# Autodesk Inventor assembly: ASY ANP 1490 FDS one way
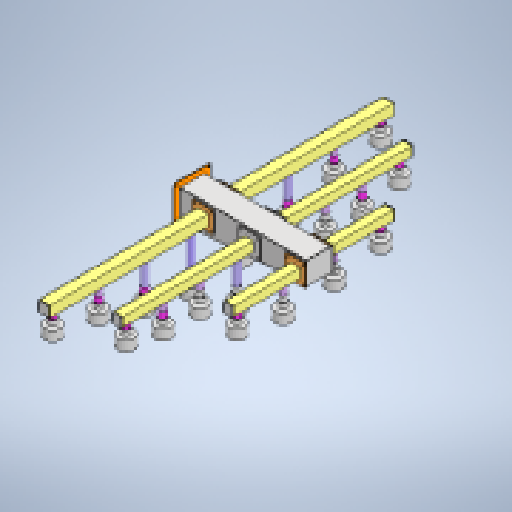
[picture p0: Inventor's stored thumbnail of the model, 512x512]
Saved by Autodesk Inventor 2025.3 (Build 293356030, 356C)
## iProperties
Created: 2025-07-22
Part Number: ASY ANP 1490 FDS one way
Document SubType Name: Assembly
Designer: admin
Stock Number: 20x40
Author: admin
## Documents named in this file (8)
- C:\Users\admin\Yandex.Disk\home pc\Inventor\ANP--Antipayuta\FDS 1400\ASY ANP 1490 FDS one way.iam
- C:\Users\admin\Yandex.Disk\home pc\Inventor\ANP--Antipayuta\FDS 1400\ANP 1422 BOTTOM FDS diameter way up.ipt
- C:\Users\admin\Yandex.Disk\home pc\Inventor\ANP--Antipayuta\FDS 1400\ANP 1421 FDS Diam way flange 1.ipt
- C:\Users\admin\Yandex.Disk\home pc\Inventor\ANP--Antipayuta\FDS 1400\ANP 1423 BOTTOM FDS diameter way down.ipt
- C:\Users\admin\Yandex.Disk\home pc\Inventor\ANP--Antipayuta\FDS 1400\ASY ANP 1425 FDS way 5.iam
- C:\Users\admin\Yandex.Disk\home pc\Inventor\ANP--Antipayuta\FDS 1400\ASY ANP 1426 FDS way 6.iam
- C:\Users\admin\Yandex.Disk\home pc\Inventor\ANP--Antipayuta\FDS 1400\ASY ANP 1427 FDS way 7.iam
- C:\Users\admin\Yandex.Disk\home pc\Inventor\ANP--Antipayuta\FDS 1400\ANP 1424 FDS diam way cup.ipt
## Components (10 placed, 10 different names)
1. ANP 1422 BOTTOM FDS diameter way up.ipt:1 — Rigid:21, Rigid:25, Rigid:26
2. ANP 1421 FDS Diam way flange 1.ipt:1
3. ANP 1423 BOTTOM FDS diameter way down.ipt:1 — Rigid:18, Rigid:22, Rigid:27, Rotational:1
4. ASY ANP 1425 FDS way 5.iam:1 [sub-assembly] — Rigid:21
5. ASY ANP 1426 FDS way 6.iam:1 [sub-assembly] — Rigid:25
6. ASY ANP 1427 FDS way 7.iam:1 [sub-assembly] — Rigid:26
7. ANP 1424 FDS diam way cup.ipt:1 — Rigid:18
8. ASY ANP 1425 FDS way 5:2 [sub-assembly] — Rigid:22
9. ASY ANP 1426 FDS way 6:2 [sub-assembly] — Rigid:27
10. ASY ANP 1427 FDS way 7:2 [sub-assembly] — Rotational:1
## Relationships (13: WeldJoint 6, Mate 3, Flush 3, RevoluteJoint 1)
- [Mate]: ANP 1422 BOTTOM FDS diameter way up.ipt:1 ↔ ANP 1421 FDS Diam way flange 1.ipt:1
- [Flush]: ANP 1422 BOTTOM FDS diameter way up.ipt:1 ↔ ANP 1421 FDS Diam way flange 1.ipt:1
- [Flush]: ANP 1422 BOTTOM FDS diameter way up.ipt:1 ↔ ANP 1421 FDS Diam way flange 1.ipt:1
- [Mate]: ANP 1421 FDS Diam way flange 1.ipt:1 ↔ ANP 1423 BOTTOM FDS diameter way down.ipt:1
- [Flush]: ANP 1421 FDS Diam way flange 1.ipt:1 ↔ ANP 1423 BOTTOM FDS diameter way down.ipt:1
- [Mate]: ANP 1422 BOTTOM FDS diameter way up.ipt:1 ↔ ANP 1423 BOTTOM FDS diameter way down.ipt:1
- Rigid:18 [WeldJoint]: ANP 1423 BOTTOM FDS diameter way down.ipt:1 ↔ ANP 1424 FDS diam way cup.ipt:1
- Rigid:21 [WeldJoint]: ANP 1422 BOTTOM FDS diameter way up.ipt:1 ↔ ASY ANP 1425 FDS way 5.iam:1
- Rigid:22 [WeldJoint]: ANP 1423 BOTTOM FDS diameter way down.ipt:1 ↔ ASY ANP 1425 FDS way 5:2
- Rigid:25 [WeldJoint]: ANP 1422 BOTTOM FDS diameter way up.ipt:1 ↔ ASY ANP 1426 FDS way 6.iam:1
- Rigid:26 [WeldJoint]: ANP 1422 BOTTOM FDS diameter way up.ipt:1 ↔ ASY ANP 1427 FDS way 7.iam:1
- Rigid:27 [WeldJoint]: ANP 1423 BOTTOM FDS diameter way down.ipt:1 ↔ ASY ANP 1426 FDS way 6:2
- Rotational:1 [RevoluteJoint]: ANP 1423 BOTTOM FDS diameter way down.ipt:1 ↔ ASY ANP 1427 FDS way 7:2
